# Autodesk Inventor assembly: rotarynozzle_Left
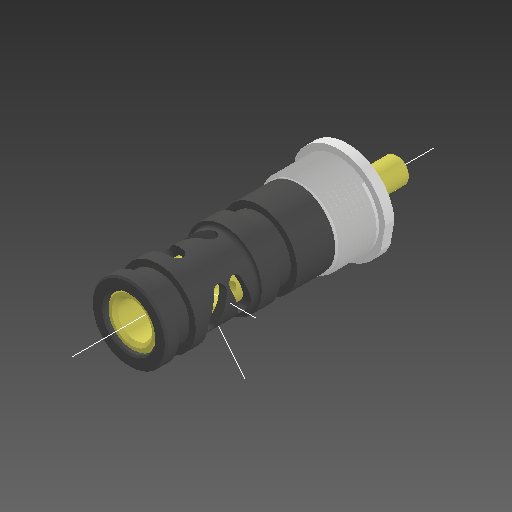
[picture p0: Inventor's stored thumbnail of the model, 512x512]
Saved by Autodesk Inventor 2021 (Build 250183000, 183)
## iProperties
Created: 2024-02-18
Part Number: rotarynozzle_Left
Document SubType Name: Assembly
Designer: top10
Author: top10
## Documents named in this file (5)
- D:\Files\Graduation Project\V4_manfoulid\Workspaces\Workspace\R_nozzle\Left\rotarynozzle_Left.iam
- D:\Files\Graduation Project\V4_manfoulid\Workspaces\Workspace\R_nozzle\Left\outer_sleeve_Left.ipt
- D:\Files\Graduation Project\V4_manfoulid\Workspaces\Workspace\R_nozzle\Left\iner_sleeve_Left.ipt
- D:\Files\Graduation Project\V4_manfoulid\Workspaces\Workspace\R_nozzle\Left\endcap_Left.ipt
- D:\Files\Graduation Project\V4_manfoulid\Workspaces\Workspace\R_nozzle\Left\bearing494_Left.ipt
## Components (4 placed, 4 different names)
1. outer_sleeve_Left:1 — Mate:10, Mate:2, Mate:1, Mate:8, Mate:5, Angle:1
2. iner_sleeve_Left:1 — Mate:10, Mate:2, Mate:3, Mate:9, Mate:4, Angle:1
3. endcap_Left:1 — Mate:3, Mate:8
4. bearing494_Left:1 — Mate:9, Mate:5, Mate:4
## Relationships (9: Mate 8, Angle 1)
- Mate:10: outer_sleeve_Left:1 ↔ iner_sleeve_Left:1
- Mate:2: outer_sleeve_Left:1 ↔ iner_sleeve_Left:1
- Mate:1: outer_sleeve_Left:1
- Mate:3: iner_sleeve_Left:1 ↔ endcap_Left:1
- Mate:8: outer_sleeve_Left:1 ↔ endcap_Left:1
- Mate:9: iner_sleeve_Left:1 ↔ bearing494_Left:1
- Mate:5: outer_sleeve_Left:1 ↔ bearing494_Left:1
- Mate:4: iner_sleeve_Left:1 ↔ bearing494_Left:1
- Angle:1 (-20 deg): outer_sleeve_Left:1 ↔ iner_sleeve_Left:1
